# Autodesk Inventor assembly: kinematicassembly
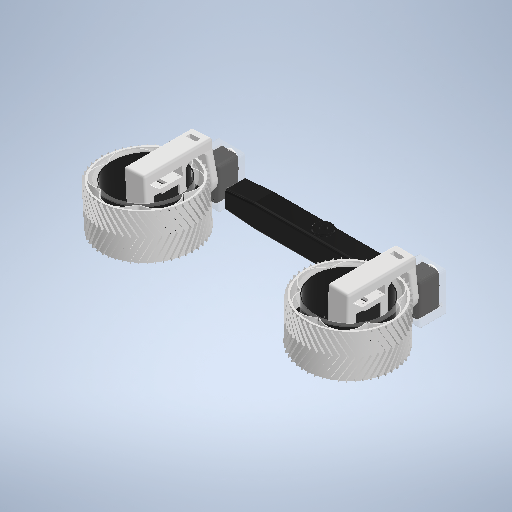
[picture p0: Inventor's stored thumbnail of the model, 512x512]
Saved by Autodesk Inventor 2025.3 (Build 293356000, 356)
## iProperties
Created: 2026-05-08
Part Number: kinematicassembly
Document SubType Name: Assembly
Designer: ksawe
Author: ksawe
## Documents named in this file (6)
- C:\Users\ksawe\OneDrive\Pulpit\Exomy v1\wersja3\kinematicassembly.iam
- C:\Users\ksawe\OneDrive\Pulpit\Exomy v1\wersja3\pret_handler_v2.ipt
- C:\Users\ksawe\OneDrive\Pulpit\Exomy v1\wersja3\basket.ipt
- C:\Users\ksawe\OneDrive\Pulpit\Exomy v1\wersja3\basketlewy.ipt
- C:\Users\ksawe\OneDrive\Pulpit\Exomy v1\wersja3\serwo.iam
- C:\Users\ksawe\OneDrive\Pulpit\Exomy v1\wersja3\modul_napedowy.iam
## Components (7 placed, 5 different names)
1. pret_handler_v2:1 — Rigid:1, Rigid:2
2. basket:1 — Rigid:2, Rigid:3
3. basketlewy:1 — Rigid:1, Rigid:4
4. serwo:1 [sub-assembly] — Rigid:3, Rigid:6
5. serwo:2 [sub-assembly] — Rigid:4, Rigid:5
6. modul_napedowy:1 [sub-assembly] — Rigid:5
7. modul_napedowy:2 [sub-assembly] — Rigid:6
## Relationships (6: WeldJoint 6)
- Rigid:1 [WeldJoint]: pret_handler_v2:1 ↔ basketlewy:1
- Rigid:2 [WeldJoint]: pret_handler_v2:1 ↔ basket:1
- Rigid:3 [WeldJoint] (1 mm): basket:1 ↔ serwo:1
- Rigid:4 [WeldJoint] (1 mm): basketlewy:1 ↔ serwo:2
- Rigid:5 [WeldJoint]: serwo:2 ↔ modul_napedowy:1
- Rigid:6 [WeldJoint]: serwo:1 ↔ modul_napedowy:2
## Named parameters: sa_0 = 5000, sa_1 = 5000
note: some values were not read from the file. Shown as the stored number, unit unknown: "sa_0", "sa_1".
